# Autodesk Inventor assembly: COTS_IGUS_045_Series_Cable_Chain
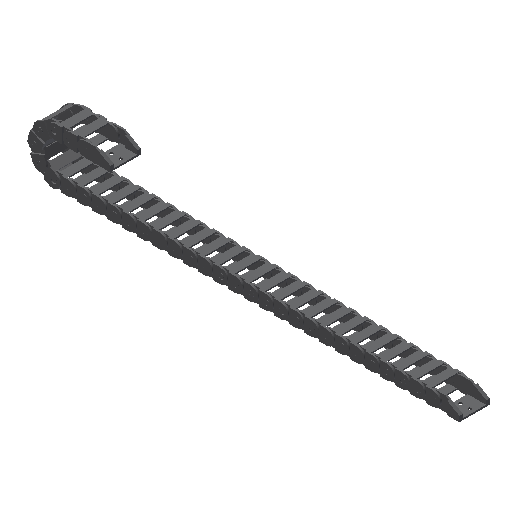
[picture p0: Inventor's stored thumbnail of the model, 512x512]
Saved by Autodesk Inventor 2026.1 (Build 301233000, 233)
## iProperties
Created: 2016-06-22
Part Number: COTS_IGUS_045_Series_Cable_Chain
Material: Ogólny
Document SubType Name: Assembly
Designer: Andrzej
Mass: 40.7133 g
Surface Area: 689.33 cm^2
Volume: 40.7133 cm^3
Density: 1 g/cm^3
Author: Andrzej
## Documents named in this file (5)
- C:\Users\Andrzej\OneDrive\_DRIVE_SYNCH_FILES\__ BYTECHLAB PROJECTS\MECH - FDM 3D Printer - RAPTOR-360\MCAD\1_REV1\__COTS_PARTS\COTS_IGUS_045_Series_Cable_Chain\COTS_IGUS_045_Series_Cable_Chain.iam
- C:\Users\Andrzej\OneDrive\_DRIVE_SYNCH_FILES\__ BYTECHLAB PROJECTS\MECH - FDM 3D Printer - RAPTOR-360\MCAD\1_REV1\__COTS_PARTS\COTS_IGUS_045_Series_Cable_Chain\0.39m 045.20.018.0_1.ipt
- C:\Users\Andrzej\OneDrive\_DRIVE_SYNCH_FILES\__ BYTECHLAB PROJECTS\MECH - FDM 3D Printer - RAPTOR-360\MCAD\1_REV1\__COTS_PARTS\COTS_IGUS_045_Series_Cable_Chain\0.39m 045.20.018.0_2.ipt
- C:\Users\Andrzej\OneDrive\_DRIVE_SYNCH_FILES\__ BYTECHLAB PROJECTS\MECH - FDM 3D Printer - RAPTOR-360\MCAD\1_REV1\__COTS_PARTS\COTS_IGUS_045_Series_Cable_Chain\Chain _skeleton.ipt
- C:\Users\Andrzej\OneDrive\_DRIVE_SYNCH_FILES\__ BYTECHLAB PROJECTS\MECH - FDM 3D Printer - RAPTOR-360\MCAD\1_REV1\__COTS_PARTS\COTS_IGUS_045_Series_Cable_Chain\0.39m 045.20.018.0_3.ipt
## Components (34 placed, 4 different names)
1. 0.39m 045.20.018.0_1:1 — Równoległy:1, Kąt:1, Wstaw:1, Kąt:2
2. 0.39m 045.20.018.0_2:1 — Równoległy:1, Kąt:1, Równoległy:2, Równoległy:3, Równoległy:4
3. Chain _skeleton:1 — Równoległy:2, Równoległy:3, Równoległy:4
4. 0.39m 045.20.018.0_3:1 — Wstaw:1, Kąt:2
5. 0.39m 045.20.018.0_3:2
6. 0.39m 045.20.018.0_3:3
7. 0.39m 045.20.018.0_3:4
8. 0.39m 045.20.018.0_3:5
9. 0.39m 045.20.018.0_3:6
10. 0.39m 045.20.018.0_3:7
11. 0.39m 045.20.018.0_3:8
12. 0.39m 045.20.018.0_3:9
13. 0.39m 045.20.018.0_3:10
14. 0.39m 045.20.018.0_3:11
15. 0.39m 045.20.018.0_3:12
16. 0.39m 045.20.018.0_3:13
17. 0.39m 045.20.018.0_3:14
18. 0.39m 045.20.018.0_3:15
19. 0.39m 045.20.018.0_3:16
20. 0.39m 045.20.018.0_3:17
21. 0.39m 045.20.018.0_3:18
22. 0.39m 045.20.018.0_3:19
23. 0.39m 045.20.018.0_3:20
24. 0.39m 045.20.018.0_3:21
25. 0.39m 045.20.018.0_3:22
26. 0.39m 045.20.018.0_3:23
27. 0.39m 045.20.018.0_3:24
28. 0.39m 045.20.018.0_3:25
29. 0.39m 045.20.018.0_3:26
30. 0.39m 045.20.018.0_3:27
31. 0.39m 045.20.018.0_3:28
32. 0.39m 045.20.018.0_3:29
33. 0.39m 045.20.018.0_3:30
34. 0.39m 045.20.018.0_3:31
## Component patterns: (31 elements, first: 0.39m 045.20.018.0_3:1)
## Relationships (7: Flush 4, Angle 2, Insert 1)
- Równoległy:1 [Flush]: 0.39m 045.20.018.0_1:1 ↔ 0.39m 045.20.018.0_2:1
- Kąt:1 [Angle] (0 deg): 0.39m 045.20.018.0_1:1 ↔ 0.39m 045.20.018.0_2:1
- Równoległy:2 [Flush]: 0.39m 045.20.018.0_2:1 ↔ Chain _skeleton:1
- Równoległy:3 [Flush]: 0.39m 045.20.018.0_2:1 ↔ Chain _skeleton:1
- Równoległy:4 [Flush]: 0.39m 045.20.018.0_2:1 ↔ Chain _skeleton:1
- Wstaw:1 [Insert]: 0.39m 045.20.018.0_1:1 ↔ 0.39m 045.20.018.0_3:1
- Kąt:2 [Angle] (0 deg): 0.39m 045.20.018.0_1:1 ↔ 0.39m 045.20.018.0_3:1
